# Autodesk Inventor assembly: KNEE_DRIVER_ASM
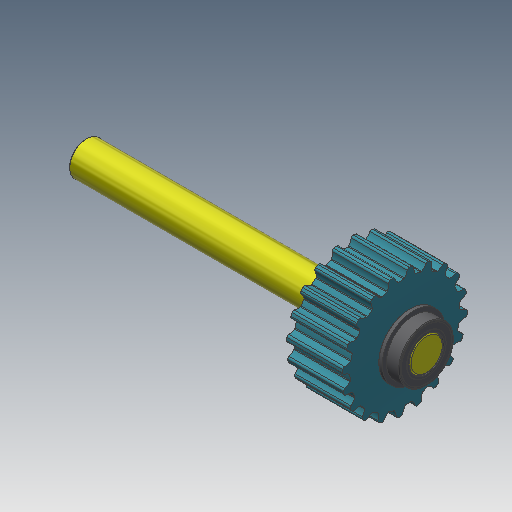
[picture p0: Inventor's stored thumbnail of the model, 512x512]
Saved by Autodesk Inventor 2019.4 (Build 234330000, 330)
## iProperties
Created: 2019-11-12
Part Number: KNEE_DRIVER_ASM
Material: 一般
Document SubType Name: Assembly
Designer: y6tada
Author: y6tada
## Documents named in this file (4)
- C:\Workspace\Yuni9\Inventor\Asm\UPPER_LEG\KNEE_DRIVER_ASM.iam
- C:\Workspace\Yuni9\Inventor\Asm\TIMING_PULLEY\TIMING_BELT_P20.ipt
- C:\Workspace\Yuni9\Inventor\Asm\UPPER_LEG\KNEE_DRIVER_SHAFT.ipt
- C:\Workspace\Yuni9\Inventor\Ref\NSK Bearing\NSK_RB_MF85ZZ\MF85ZZ.iam
## Components (3 placed, 3 different names)
1. TIMING_BELT_P20:1 — メイト:3
2. KNEE_DRIVER_SHAFT:1 — メイト:1, メイト:2, メイト:3, メイト:4, フラッシュ:1
3. MF85ZZ:1 [sub-assembly] — メイト:4, フラッシュ:1
## Relationships (5: Mate 4, Flush 1)
- メイト:1 [Mate]: KNEE_DRIVER_SHAFT:1
- メイト:2 [Mate]: KNEE_DRIVER_SHAFT:1
- メイト:3 [Mate]: TIMING_BELT_P20:1 ↔ KNEE_DRIVER_SHAFT:1
- メイト:4 [Mate]: KNEE_DRIVER_SHAFT:1 ↔ MF85ZZ:1
- フラッシュ:1 [Flush]: KNEE_DRIVER_SHAFT:1 ↔ MF85ZZ:1
